# Autodesk Inventor assembly: foreuse
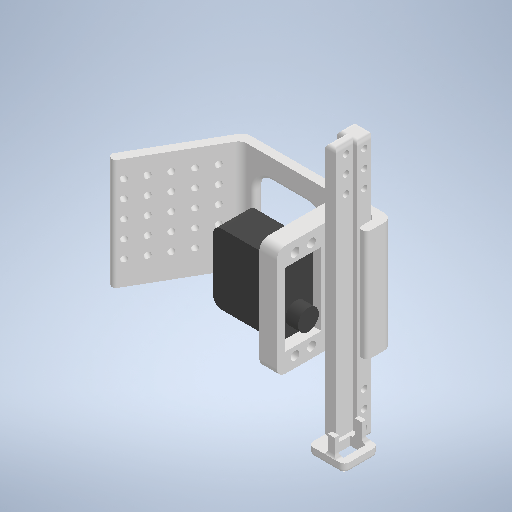
[picture p0: Inventor's stored thumbnail of the model, 512x512]
Saved by Autodesk Inventor 2025 (Build 290162000, 162)
## iProperties
Created: 2024-09-30
Part Number: foreuse
Document SubType Name: Assembly
Designer: chass
Author: chass
## Documents named in this file (4)
- C:\Users\chass\Documents\AREM\CdR-2024\Robot\Modelisations-3D\Modèles3D_Actionneur_robot_cdr\Tourneur_de_panneaux_solaires\foreuse.iam
- C:\Users\chass\Documents\AREM\CdR-2024\Robot\Modelisations-3D\Modèles3D_Actionneur_robot_cdr\Tourneur_de_panneaux_solaires\doigt_FDS_foreuse.ipt
- C:\Users\chass\Documents\AREM\CdR-2024\Robot\Modelisations-3D\Modèles3D_Actionneur_robot_cdr\Tourneur_de_panneaux_solaires\Support2.ipt
- C:\Users\chass\Documents\AREM\Hackathon_2024\Modeles_3D\servomoteur_roues.ipt
## Components (3 placed, 3 different names)
1. doigt_FDS_foreuse:1 — Placage:1, Placage:2
2. Support2:1 — Placage:1, Placage:2, Placage:3, Placage:4, Placage:5
3. servomoteur_roues:1 — Placage:3, Placage:4, Placage:5
## Relationships (5: Mate 5)
- Placage:1 [Mate]: doigt_FDS_foreuse:1 ↔ Support2:1
- Placage:2 [Mate]: doigt_FDS_foreuse:1 ↔ Support2:1
- Placage:3 [Mate]: Support2:1 ↔ servomoteur_roues:1
- Placage:4 [Mate]: Support2:1 ↔ servomoteur_roues:1
- Placage:5 [Mate]: Support2:1 ↔ servomoteur_roues:1
